# Autodesk Inventor assembly: Kook Assembly
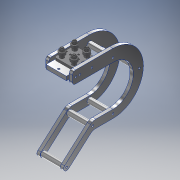
[picture p0: Inventor's stored thumbnail of the model, 180x180]
Saved by Autodesk Inventor 2019.4 (Build 234330000, 330)
## iProperties
Created: 2020-03-10
Part Number: Kook Assembly
Document SubType Name: Assembly
Designer: admin
Author: admin
## Documents named in this file (5)
- C:\Users\admin\Desktop\FRC 2020 Engineering\GitHub\7738-2020\Robot V2\Hook\Kook Assembly.iam
- C:\Users\admin\Desktop\FRC 2020 Engineering\GitHub\7738-2020\7738-Adjuster\Mini V Gantry Kit.iam
- C:\Users\admin\Desktop\FRC 2020 Engineering\GitHub\7738-2020\Robot V2\Hook\Hook Part.ipt
- C:\Users\admin\Desktop\FRC 2020 Engineering\GitHub\7738-2020\Robot V2\Hook\Hook Plate.ipt
- C:\Users\admin\Desktop\FRC 2020 Engineering\GitHub\7738-2020\Robot V2\Hook\Hook Plate Spacer.ipt
## Components (9 placed, 4 different names)
1. Hook Part:1 — Mate:4, Mate:5, Mate:6, Mate:7, Mate:8, Mate:9, Mate:18, Mate:19, Mate:20
2. Hook Plate:1 — Mate:4, Mate:5, Mate:6, Mate:10, Mate:11, Mate:12, Mate:13
3. Hook Plate:2 — Mate:7, Mate:8, Mate:9, Mate:14, Mate:15, Mate:16, Mate:17, Mate:21, Mate:22
4. Hook Plate Spacer:1 — Mate:10, Mate:14
5. Hook Plate Spacer:2 — Mate:11, Mate:15
6. Hook Plate Spacer:3 — Mate:13, Mate:17
7. Hook Plate Spacer:4 — Mate:12, Mate:16
8. Mini V Gantry Kit:1 [sub-assembly] — Mate:18, Mate:19, Mate:20
9. Hook Plate Spacer:5 — Mate:21, Mate:22
## Relationships (19: Mate 19)
- Mate:4: Hook Part:1 ↔ Hook Plate:1
- Mate:5: Hook Part:1 ↔ Hook Plate:1
- Mate:6: Hook Part:1 ↔ Hook Plate:1
- Mate:7: Hook Part:1 ↔ Hook Plate:2
- Mate:8: Hook Part:1 ↔ Hook Plate:2
- Mate:9: Hook Part:1 ↔ Hook Plate:2
- Mate:10: Hook Plate:1 ↔ Hook Plate Spacer:1
- Mate:11: Hook Plate:1 ↔ Hook Plate Spacer:2
- Mate:12: Hook Plate:1 ↔ Hook Plate Spacer:4
- Mate:13: Hook Plate:1 ↔ Hook Plate Spacer:3
- Mate:14: Hook Plate:2 ↔ Hook Plate Spacer:1
- Mate:15: Hook Plate:2 ↔ Hook Plate Spacer:2
- Mate:16: Hook Plate:2 ↔ Hook Plate Spacer:4
- Mate:17: Hook Plate:2 ↔ Hook Plate Spacer:3
- Mate:18: Hook Part:1 ↔ Mini V Gantry Kit:1
- Mate:19: Hook Part:1 ↔ Mini V Gantry Kit:1
- Mate:20: Hook Part:1 ↔ Mini V Gantry Kit:1
- Mate:21: Hook Plate:2 ↔ Hook Plate Spacer:5
- Mate:22: Hook Plate:2 ↔ Hook Plate Spacer:5
